# Autodesk Inventor assembly: WCP-0155 2 Motor Flipped Gearbox
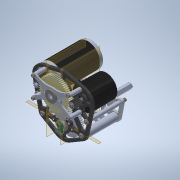
[picture p0: Inventor's stored thumbnail of the model, 180x180]
Saved by Autodesk Inventor 2020 (Build 240168000, 168)
## iProperties
Created: 2019-01-05
Part Number: WCP-0155 2 Motor Flipped Gearbox
Description: STEP AP214
Document SubType Name: Assembly
Designer: Alex
Mass: 1434.74 g
Surface Area: 3117.27 cm^2
Volume: 1434.74 cm^3
Density: 1 g/cm^3
Sending System: SolidWorks 2018
Preprocessor: SwSTEP 2.0
Title: WCP-0155 Rev1 - WCP 3 Motor Flipped Gearbox (SS).STEP
Revision Number: ANY
## Documents named in this file (31)
- C:\Users\turnm\Documents\GrabCAD\Infinite Recharge 2020\Build season\WCP-0155 2 Motor Flipped Gearbox.iam
- C:\Users\turnm\Documents\GrabCAD\Infinite Recharge 2020\Build season\DGB STEP\WCP-0155-002 Rev1_MIR.ipt
- C:\Users\turnm\Documents\GrabCAD\Infinite Recharge 2020\Build season\DGB STEP\WCP-0155-006 Rev1_MIR.ipt
- C:\Users\turnm\Documents\GrabCAD\Infinite Recharge 2020\Build season\DGB STEP\WCP-0155-003 Rev1_MIR.ipt
- C:\Users\turnm\Documents\GrabCAD\Infinite Recharge 2020\Build season\DGB STEP\WCP-0155-004 Rev1_MIR.ipt
- C:\Users\turnm\Documents\GrabCAD\Infinite Recharge 2020\Build season\DGB STEP\WCP-0155-005 Rev1_MIR.ipt
- C:\Users\turnm\Documents\GrabCAD\Infinite Recharge 2020\Build season\DGB STEP\WCP-0155-007 Rev1_MIR.ipt
- C:\Users\turnm\Documents\GrabCAD\Infinite Recharge 2020\Build season\DGB STEP\WCP-0155-008 Rev1_MIR.ipt
- C:\Users\turnm\Documents\GrabCAD\Infinite Recharge 2020\Build season\DGB STEP\WCP-0155-009 Rev1_MIR.ipt
- C:\Users\turnm\Documents\GrabCAD\Infinite Recharge 2020\Build season\DGB STEP\WCP-0155-010 Rev1_MIR.ipt
- C:\Users\turnm\Documents\GrabCAD\Infinite Recharge 2020\Build season\DGB STEP\WCP-0155-012 Rev1_MIR.ipt
- C:\Users\turnm\Documents\GrabCAD\Infinite Recharge 2020\Build season\DGB STEP\217-2731_0_500_flanged_bearing_MIR.ipt
- C:\Users\turnm\Documents\GrabCAD\Infinite Recharge 2020\Build season\DGB STEP\217-4006_0_500_flanged_thunderhex_bearing_MIR.ipt
- C:\Users\turnm\Documents\GrabCAD\Infinite Recharge 2020\Build season\DGB STEP\WCP-0112 Rev1_MIR.ipt
- C:\Users\turnm\Documents\GrabCAD\Infinite Recharge 2020\Build season\DGB STEP\217-3099_12T_CIM_MIR.ipt
- C:\Users\turnm\Documents\GrabCAD\Infinite Recharge 2020\Build season\DGB STEP\217-3574_60T_500_hex_MIR.ipt
- C:\Users\turnm\Documents\GrabCAD\Infinite Recharge 2020\Build season\DGB STEP\217-2708_40T_500_hex_MIR.ipt
- C:\Users\turnm\Documents\GrabCAD\Infinite Recharge 2020\Build season\DGB STEP\217-3572_50T_500_hex_MIR.ipt
- C:\Users\turnm\Documents\GrabCAD\Infinite Recharge 2020\Build season\DGB STEP\217-2000_CIM_MIR.ipt
- C:\Users\turnm\Documents\GrabCAD\Infinite Recharge 2020\Build season\DGB STEP\NFS-0003_SHCS_#10-32_4_000L_Default_As Machined__MIR.ipt
- C:\Users\turnm\Documents\GrabCAD\Infinite Recharge 2020\Build season\DGB STEP\NFS-0018_SHCS_#10-32_1_750L_Default_As Machined__MIR.ipt
- C:\Users\turnm\Documents\GrabCAD\Infinite Recharge 2020\Build season\DGB STEP\NFS-0002_BHCS_#10-32_0_250L_Default_As Machined__MIR.ipt
- C:\Users\turnm\Documents\GrabCAD\Infinite Recharge 2020\Build season\DGB STEP\NFS-0010_#10-32_thin_locknut_Default_As Machined__MIR.ipt
- C:\Users\turnm\Documents\GrabCAD\Infinite Recharge 2020\Build season\DGB STEP\NFS-0009_0_500_snapring_97633A200_MIR.ipt
- C:\Users\turnm\Documents\GrabCAD\Infinite Recharge 2020\Build season\DGB STEP\NFS-0031_8mm_push_nut_92133A109_MIR.ipt
- C:\Users\turnm\Documents\GrabCAD\Infinite Recharge 2020\Build season\DGB STEP\NFS-0035_Machine_Key_2x2mm_20mmL_96717A075_MIR.ipt
- C:\Users\turnm\Documents\GrabCAD\Infinite Recharge 2020\Build season\DGB STEP\NFS-0036_Wave_Washer_9714K33_MIR.ipt
- C:\Users\turnm\Documents\GrabCAD\Infinite Recharge 2020\Build season\DGB STEP\0_500_L_500_hex_spacer_217-3261_MIR.ipt
- C:\Users\turnm\Documents\GrabCAD\Infinite Recharge 2020\Brainstorming\WCP-0249-001 Rev1_MIR.ipt
- C:\Users\turnm\Documents\GrabCAD\Infinite Recharge 2020\Build season\RevRobotics\REV-21-1650 Neo Motor.ipt
- C:\Users\turnm\Documents\GrabCAD\Infinite Recharge 2020\Build season\EncoderCAD\EncoderAssembly.iam
## Components (55 placed, 30 different names)
1. WCP-0155-002 Rev1_MIR:1 — Mate:21, Mate:20, Mate:22, Mate:11, Mate:10, Mate:13, Mate:12, Insert:4, Insert:3, Angle:2
2. WCP-0155-006 Rev1_MIR:1
3. WCP-0155-003 Rev1_MIR:1
4. WCP-0155-004 Rev1_MIR:1 — Mate:29, Flush:2
5. WCP-0155-005 Rev1_MIR:1
6. WCP-0155-007 Rev1_MIR:1 — Mate:21, Mate:26
7. WCP-0155-007 Rev1_MIR:2 — Mate:20, Mate:24, Mate:19, Mate:18
8. WCP-0155-006 Rev1_MIR:2 — Mate:22, Mate:16, Mate:17
9. WCP-0155-008 Rev1_MIR:1
10. WCP-0155-008 Rev1_MIR:2 — Mate:4
11. WCP-0155-008 Rev1_MIR:3 — Mate:5
12. WCP-0155-008 Rev1_MIR:4
13. WCP-0155-009 Rev1_MIR:1
14. WCP-0155-010 Rev1_MIR:1
15. WCP-0155-012 Rev1_MIR:1 — Mate:3, Mate:2, Mate:9, Angle:1, Mate:33
16. 217-2731_0_500_flanged_bearing_MIR:1
17. 217-2731_0_500_flanged_bearing_MIR:2
18. 217-2731_0_500_flanged_bearing_MIR:3
19. 217-2731_0_500_flanged_bearing_MIR:4 — Mate:29, Flush:2, Insert:3
20. 217-4006_0_500_flanged_thunderhex_bearing_MIR:1
21. WCP-0112 Rev1_MIR:1
22. WCP-0112 Rev1_MIR:2 — Flush:1
23. 217-3099_12T_CIM_MIR:1
24. 217-3099_12T_CIM_MIR:3
25. 217-3574_60T_500_hex_MIR:1
26. 217-2708_40T_500_hex_MIR:1
27. 217-3572_50T_500_hex_MIR:1 — Flush:1, Mate:3, Mate:2, Mate:8
28. 217-2000_CIM_MIR:1 — Insert:1
29. NFS-0003_SHCS_#10-32_4_000L_Default_As Machined__MIR:1 — Mate:16, Mate:11, Mate:10, Mate:14
30. NFS-0003_SHCS_#10-32_4_000L_Default_As Machined__MIR:2 — Mate:13, Mate:12, Mate:28
31. NFS-0018_SHCS_#10-32_1_750L_Default_As Machined__MIR:1
32. NFS-0018_SHCS_#10-32_1_750L_Default_As Machined__MIR:2
33. NFS-0018_SHCS_#10-32_1_750L_Default_As Machined__MIR:3 — Mate:31
34. NFS-0018_SHCS_#10-32_1_750L_Default_As Machined__MIR:4 — Mate:30
35. NFS-0002_BHCS_#10-32_0_250L_Default_As Machined__MIR:1
36. NFS-0002_BHCS_#10-32_0_250L_Default_As Machined__MIR:2
37. NFS-0002_BHCS_#10-32_0_250L_Default_As Machined__MIR:3
38. NFS-0002_BHCS_#10-32_0_250L_Default_As Machined__MIR:4 — Insert:4
39. NFS-0010_#10-32_thin_locknut_Default_As Machined__MIR:1 — Mate:28, Mate:27
40. NFS-0010_#10-32_thin_locknut_Default_As Machined__MIR:2 — Mate:26, Mate:25
41. NFS-0010_#10-32_thin_locknut_Default_As Machined__MIR:3 — Mate:24, Mate:23
42. NFS-0010_#10-32_thin_locknut_Default_As Machined__MIR:4 — Mate:14, Mate:15
43. NFS-0009_0_500_snapring_97633A200_MIR:1
44. NFS-0009_0_500_snapring_97633A200_MIR:2 — Mate:9
45. NFS-0031_8mm_push_nut_92133A109_MIR:1
46. NFS-0031_8mm_push_nut_92133A109_MIR:2
47. NFS-0031_8mm_push_nut_92133A109_MIR:3
48. NFS-0031_8mm_push_nut_92133A109_MIR:4
49. NFS-0035_Machine_Key_2x2mm_20mmL_96717A075_MIR:2
50. NFS-0035_Machine_Key_2x2mm_20mmL_96717A075_MIR:3
51. NFS-0036_Wave_Washer_9714K33_MIR:1
52. 0_500_L_500_hex_spacer_217-3261_MIR:1
53. WCP-0249-001 Rev1_MIR:1 — Mate:27, Mate:25, Mate:23, Mate:19, Mate:18, Mate:17, Mate:15, Mate:8, Insert:1, Mate:32, Tangent:1, Mate:34, Angle:3
54. REV-21-1650 Neo Motor:1 — Mate:30, Mate:31, Mate:32
55. EncoderAssembly:1 [sub-assembly] — Mate:33, Mate:35, Mate:36
## Relationships (45: Mate 35, Flush 3, Insert 3, Angle 3, Tangent 1)
- Mate:21: WCP-0155-002 Rev1_MIR:1 ↔ WCP-0155-007 Rev1_MIR:1
- Mate:20: WCP-0155-002 Rev1_MIR:1 ↔ WCP-0155-007 Rev1_MIR:2
- Mate:22: WCP-0155-002 Rev1_MIR:1 ↔ WCP-0155-006 Rev1_MIR:2
- Flush:1: WCP-0112 Rev1_MIR:2 ↔ 217-3572_50T_500_hex_MIR:1
- Mate:3: WCP-0155-012 Rev1_MIR:1 ↔ 217-3572_50T_500_hex_MIR:1
- Mate:2: WCP-0155-012 Rev1_MIR:1 ↔ 217-3572_50T_500_hex_MIR:1
- Mate:16: WCP-0155-006 Rev1_MIR:2 ↔ NFS-0003_SHCS_#10-32_4_000L_Default_As Machined__MIR:1
- Mate:11 (3.175 mm): WCP-0155-002 Rev1_MIR:1 ↔ NFS-0003_SHCS_#10-32_4_000L_Default_As Machined__MIR:1
- Mate:10: WCP-0155-002 Rev1_MIR:1 ↔ NFS-0003_SHCS_#10-32_4_000L_Default_As Machined__MIR:1
- Mate:13 (3.175 mm): WCP-0155-002 Rev1_MIR:1 ↔ NFS-0003_SHCS_#10-32_4_000L_Default_As Machined__MIR:2
- Mate:12: WCP-0155-002 Rev1_MIR:1 ↔ NFS-0003_SHCS_#10-32_4_000L_Default_As Machined__MIR:2
- Insert:4: WCP-0155-002 Rev1_MIR:1 ↔ NFS-0002_BHCS_#10-32_0_250L_Default_As Machined__MIR:4
- Mate:28: NFS-0003_SHCS_#10-32_4_000L_Default_As Machined__MIR:2 ↔ NFS-0010_#10-32_thin_locknut_Default_As Machined__MIR:1
- Mate:26: WCP-0155-007 Rev1_MIR:1 ↔ NFS-0010_#10-32_thin_locknut_Default_As Machined__MIR:2
- Mate:24: WCP-0155-007 Rev1_MIR:2 ↔ NFS-0010_#10-32_thin_locknut_Default_As Machined__MIR:3
- Mate:14: NFS-0003_SHCS_#10-32_4_000L_Default_As Machined__MIR:1 ↔ NFS-0010_#10-32_thin_locknut_Default_As Machined__MIR:4
- Mate:9: WCP-0155-012 Rev1_MIR:1 ↔ NFS-0009_0_500_snapring_97633A200_MIR:2
- Mate:27: NFS-0010_#10-32_thin_locknut_Default_As Machined__MIR:1 ↔ WCP-0249-001 Rev1_MIR:1
- Mate:25: NFS-0010_#10-32_thin_locknut_Default_As Machined__MIR:2 ↔ WCP-0249-001 Rev1_MIR:1
- Mate:23: NFS-0010_#10-32_thin_locknut_Default_As Machined__MIR:3 ↔ WCP-0249-001 Rev1_MIR:1
- Mate:19: WCP-0155-007 Rev1_MIR:2 ↔ WCP-0249-001 Rev1_MIR:1
- Mate:18: WCP-0155-007 Rev1_MIR:2 ↔ WCP-0249-001 Rev1_MIR:1
- Mate:17: WCP-0155-006 Rev1_MIR:2 ↔ WCP-0249-001 Rev1_MIR:1
- Mate:15: NFS-0010_#10-32_thin_locknut_Default_As Machined__MIR:4 ↔ WCP-0249-001 Rev1_MIR:1
- Mate:8: 217-3572_50T_500_hex_MIR:1 ↔ WCP-0249-001 Rev1_MIR:1
- Insert:1: 217-2000_CIM_MIR:1 ↔ WCP-0249-001 Rev1_MIR:1
- Mate:4: WCP-0155-008 Rev1_MIR:2
- Mate:5: WCP-0155-008 Rev1_MIR:3
- Angle:1 (0 deg): WCP-0155-012 Rev1_MIR:1
- Mate:7
- Mate:6
- Mate:29: WCP-0155-004 Rev1_MIR:1 ↔ 217-2731_0_500_flanged_bearing_MIR:4
- Flush:2: WCP-0155-004 Rev1_MIR:1 ↔ 217-2731_0_500_flanged_bearing_MIR:4
- Insert:3: WCP-0155-002 Rev1_MIR:1 ↔ 217-2731_0_500_flanged_bearing_MIR:4
- Mate:30: NFS-0018_SHCS_#10-32_1_750L_Default_As Machined__MIR:4 ↔ REV-21-1650 Neo Motor:1
- Mate:31: NFS-0018_SHCS_#10-32_1_750L_Default_As Machined__MIR:3 ↔ REV-21-1650 Neo Motor:1
- Mate:32: WCP-0249-001 Rev1_MIR:1 ↔ REV-21-1650 Neo Motor:1
- Mate:33: WCP-0155-012 Rev1_MIR:1 ↔ EncoderAssembly:1
- Angle:2 (0 deg): WCP-0155-002 Rev1_MIR:1
- Tangent:1: WCP-0249-001 Rev1_MIR:1
- Flush:3 (36.7665 mm)
- Mate:34: WCP-0249-001 Rev1_MIR:1
- Angle:3 (0 deg): WCP-0249-001 Rev1_MIR:1
- Mate:35: EncoderAssembly:1
- Mate:36 (-19.05 mm): EncoderAssembly:1
